# Autodesk Inventor assembly: PostLensHolder_B1S_PLS3in
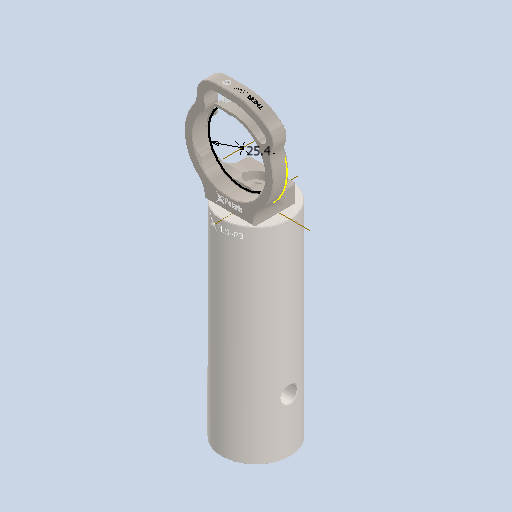
[picture p0: Inventor's stored thumbnail of the model, 512x512]
Saved by Autodesk Inventor 2024.2 (Build 282272000, 272)
## iProperties
Created: 2023-10-19
Part Number: PostLensHolder_B1S_PLS3in
Document SubType Name: Assembly
Designer: S227943
Author: S227943
## Documents named in this file (3)
- C:\Users\monolithic\Documents\GitHub\CAD\Monolith\John\ASLM_SampleScanning_Baseplate\Assembly\Components\SubAssemblies\PostLensHolder_B1S_PLS3in.iam
- C:\Users\monolithic\Documents\GitHub\CAD\Monolith\John\ASLM_SampleScanning_Baseplate\Assembly\Components\SubAssemblies\POLARIS-B1S-1inOptics.ipt
- C:\Users\monolithic\Documents\GitHub\CAD\Monolith\John\ASLM_SampleScanning_Baseplate\Assembly\Components\SubAssemblies\PLS-P3.ipt
## Components (2 placed, 2 different names)
1. POLARIS-B1S-1inOptics:1 — Mate:8, Mate:9
2. PLS-P3:1 — Mate:8, Mate:9
## Relationships (2: Mate 2)
- Mate:8: POLARIS-B1S-1inOptics:1 ↔ PLS-P3:1
- Mate:9: POLARIS-B1S-1inOptics:1 ↔ PLS-P3:1
